# Autodesk Inventor assembly: 1U CubeSat
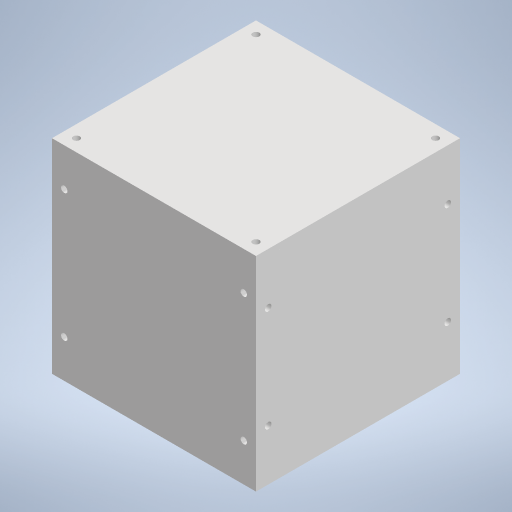
[picture p0: Inventor's stored thumbnail of the model, 512x512]
Saved by Autodesk Inventor 2023 (Build 270158000, 158)
## iProperties
Created: 2022-07-23
Part Number: 1U CubeSat
Document SubType Name: Assembly
Designer: Aditya Bansal
Author: Aditya Bansal
## Documents named in this file (6)
- C:\Users\Aditya Bansal\OneDrive - UNSW\Uni\BlueSat\1U CubeSat.iam
- C:\Users\Aditya Bansal\OneDrive - UNSW\Uni\BlueSat\BottomPlate.ipt
- C:\Users\Aditya Bansal\OneDrive - UNSW\Uni\BlueSat\VerticalStrut.ipt
- C:\Users\Aditya Bansal\OneDrive - UNSW\Uni\BlueSat\TopPlate.ipt
- C:\Users\Aditya Bansal\OneDrive - UNSW\Uni\BlueSat\FrontPanel.ipt
- C:\Users\Aditya Bansal\OneDrive - UNSW\Uni\BlueSat\SidePanel.ipt
## Components (10 placed, 5 different names)
1. BottomPlate:1 — Mate:1, Flush:1, Flush:2, Insert:1, Insert:2, Insert:3
2. VerticalStrut:1 — Mate:1, Flush:1, Flush:2, Flush:3, Insert:8, Insert:11
3. VerticalStrut:2 — Insert:1, Flush:3, Flush:4, Insert:5, Insert:7, Insert:10
4. VerticalStrut:3 — Flush:4, Insert:2, Flush:5, Insert:6, Insert:13
5. VerticalStrut:4 — Insert:3, Flush:5, Insert:4, Insert:9, Insert:12
6. TopPlate:1 — Insert:4, Insert:5
7. FrontPanel:1 — Insert:6, Insert:7
8. FrontPanel:2 — Insert:8, Insert:9
9. SidePanel:1 — Insert:10, Insert:11
10. SidePanel:2 — Insert:12, Insert:13
## Relationships (19: Insert 13, Flush 5, Mate 1)
- Mate:1: BottomPlate:1 ↔ VerticalStrut:1
- Flush:1 (3 mm): BottomPlate:1 ↔ VerticalStrut:1
- Flush:2 (3 mm): BottomPlate:1 ↔ VerticalStrut:1
- Insert:1: BottomPlate:1 ↔ VerticalStrut:2
- Flush:3: VerticalStrut:1 ↔ VerticalStrut:2
- Flush:4: VerticalStrut:2 ↔ VerticalStrut:3
- Insert:2: BottomPlate:1 ↔ VerticalStrut:3
- Insert:3: BottomPlate:1 ↔ VerticalStrut:4
- Flush:5: VerticalStrut:3 ↔ VerticalStrut:4
- Insert:4: VerticalStrut:4 ↔ TopPlate:1
- Insert:5: VerticalStrut:2 ↔ TopPlate:1
- Insert:6: VerticalStrut:3 ↔ FrontPanel:1
- Insert:7: VerticalStrut:2 ↔ FrontPanel:1
- Insert:8: VerticalStrut:1 ↔ FrontPanel:2
- Insert:9: VerticalStrut:4 ↔ FrontPanel:2
- Insert:10: VerticalStrut:2 ↔ SidePanel:1
- Insert:11: VerticalStrut:1 ↔ SidePanel:1
- Insert:12: VerticalStrut:4 ↔ SidePanel:2
- Insert:13: VerticalStrut:3 ↔ SidePanel:2
